# Autodesk Inventor assembly: ESP Moount
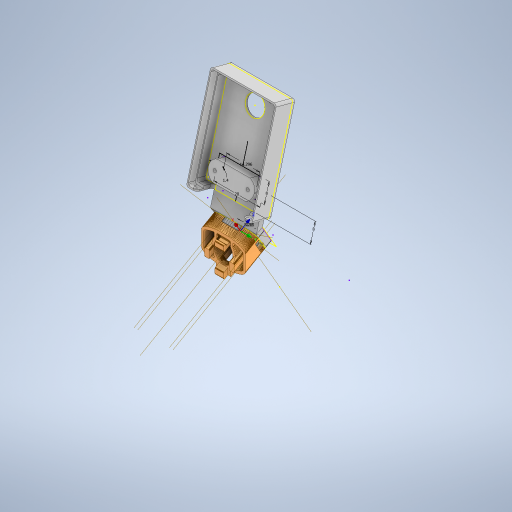
[picture p0: Inventor's stored thumbnail of the model, 512x512]
Saved by Autodesk Inventor 2023 (Build 270158000, 158)
## iProperties
Created: 2023-02-22
Part Number: ESP Moount
Document SubType Name: Assembly
Designer: tommi
Author: tommi
## Documents named in this file (4)
- C:\Users\tommi\Robot_Dog\docs\Inventor\ESP Moount.iam
- C:\Users\tommi\Documents\Inventor\Bittle Upgrades\CAM-Front-Test-V7.ipt
- C:\Users\tommi\Documents\Inventor\Bittle Upgrades\Cam-Neck conection.ipt
- C:\Users\tommi\Documents\Inventor\Bittle Upgrades\Bittle_neck_raw.ipt
## Components (3 placed, 3 different names)
1. CAM-Front-Test-V7:1 — Starr:2
2. Cam-Neck conection:1 — Starr:1, Starr:2
3. Bittle_neck_raw:1 — Starr:1
## Relationships (2: WeldJoint 2)
- Starr:1 [WeldJoint]: Cam-Neck conection:1 ↔ Bittle_neck_raw:1
- Starr:2 [WeldJoint]: CAM-Front-Test-V7:1 ↔ Cam-Neck conection:1
